# Autodesk Inventor assembly: Assembly1
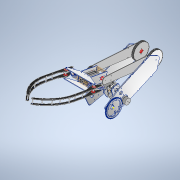
[picture p0: Inventor's stored thumbnail of the model, 180x180]
Saved by Autodesk Inventor 2021 (Build 250183000, 183)
## iProperties
Created: 2022-02-02
Part Number: Assembly1
Document SubType Name: Assembly
Designer: hirohumi
Author: hirohumi
## Documents named in this file (9)
- C:\Users\hirohumi\OneDrive\ドキュメント\ロボ研\2022NHKロボコン\R2_version1\3軸アーム\Assembly1.iam
- C:\Users\hirohumi\OneDrive\ドキュメント\ロボ研\2022NHKロボコン\R2_version1\3軸アーム\関節2_側板1.ipt
- C:\Users\hirohumi\OneDrive\ドキュメント\ロボ研\2022NHKロボコン\R2_version1\3軸アーム\プーリ_歯数60.ipt
- C:\Users\hirohumi\OneDrive\ドキュメント\ロボ研\2022NHKロボコン\R2_version1\R2_ハンド.iam
- C:\Users\hirohumi\OneDrive\ドキュメント\ロボ研\2022NHKロボコン\R2_version1\3軸アーム\関節3.iam
- C:\Users\hirohumi\OneDrive\ドキュメント\ロボ研\2022NHKロボコン\R2_version1\3軸アーム\ベアリングフランジなし.ipt
- C:\Users\hirohumi\OneDrive\ドキュメント\ロボ研\2022NHKロボコン\R2_version1\3軸アーム\ベアリングフランジ付き.ipt
- C:\Users\hirohumi\OneDrive\ドキュメント\ロボ研\2022NHKロボコン\R2_version1\3軸アーム\軸8-80.ipt
- C:\Users\hirohumi\OneDrive\ドキュメント\ロボ研\2022NHKロボコン\R2_version1\3軸アーム\関節1_プーリ2個.iam
## Components (13 placed, 8 different names)
1. R2_ハンド:1 [sub-assembly] — 挿入:1, 挿入:2, 挿入:3
2. ベアリングフランジなし:1 — 挿入:1, メイト:1, メイト:5
3. ベアリングフランジ付き:1 — 挿入:3
4. ベアリングフランジ付き:2 — 挿入:2
5. 軸8-80:1 — 挿入:4, 挿入:5, メイト:1
6. 関節2_側板1:1 — 挿入:4, 挿入:11, メイト:5
7. 関節2_側板1:2 — 挿入:5, 挿入:8, 挿入:9, メイト:3
8. プーリ_歯数60:1 — 挿入:6, 挿入:7, 挿入:8, 挿入:9
9. プーリ_歯数60:2 — 挿入:6, 挿入:7, 挿入:10
10. ベアリングフランジなし:2 — 挿入:10, メイト:6
11. ベアリングフランジ付き:3 — 挿入:11, メイト:2, メイト:3, メイト:4
12. 関節1_プーリ2個:1 [sub-assembly] — メイト:2
13. 関節3:1 [sub-assembly] — メイト:4, メイト:6
## Relationships (17: Insert 11, Mate 6)
- 挿入:1 [Insert]: R2_ハンド:1 ↔ ベアリングフランジなし:1
- 挿入:2 [Insert]: R2_ハンド:1 ↔ ベアリングフランジ付き:2
- 挿入:3 [Insert]: R2_ハンド:1 ↔ ベアリングフランジ付き:1
- 挿入:4 [Insert]: 軸8-80:1 ↔ 関節2_側板1:1
- 挿入:5 [Insert]: 軸8-80:1 ↔ 関節2_側板1:2
- 挿入:6 [Insert]: プーリ_歯数60:1 ↔ プーリ_歯数60:2
- 挿入:7 [Insert]: プーリ_歯数60:1 ↔ プーリ_歯数60:2
- 挿入:8 [Insert]: 関節2_側板1:2 ↔ プーリ_歯数60:1
- 挿入:9 [Insert]: 関節2_側板1:2 ↔ プーリ_歯数60:1
- 挿入:10 [Insert]: プーリ_歯数60:2 ↔ ベアリングフランジなし:2
- 挿入:11 [Insert]: 関節2_側板1:1 ↔ ベアリングフランジ付き:3
- メイト:1 [Mate]: ベアリングフランジなし:1 ↔ 軸8-80:1
- メイト:2 [Mate]: ベアリングフランジ付き:3 ↔ 関節1_プーリ2個:1
- メイト:3 [Mate]: 関節2_側板1:2 ↔ ベアリングフランジ付き:3
- メイト:4 [Mate]: ベアリングフランジ付き:3 ↔ 関節3:1
- メイト:5 [Mate]: ベアリングフランジなし:1 ↔ 関節2_側板1:1
- メイト:6 [Mate]: ベアリングフランジなし:2 ↔ 関節3:1
